# Autodesk Inventor assembly: Flywheels
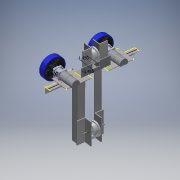
[picture p0: Inventor's stored thumbnail of the model, 180x180]
Saved by Autodesk Inventor 2017 (Build 210142000, 142)
## iProperties
Created: 2016-10-19
Part Number: Flywheels
Document SubType Name: Assembly
Designer: Aditya
Author: Aditya
## Documents named in this file (14)
- C:\Users\Aditya\Documents\GitHub\RobotuxCAD\Team Robotux 15-16 Robot Cad Assets\Flywheels.iam
- C:\Users\Aditya\Documents\GitHub\RobotuxCAD\Team Robotux 15-16 Robot Cad Assets\Flywheel w motor.iam
- C:\Users\Aditya\Documents\GitHub\RobotuxCAD\Team Robotux 15-16 Robot Cad Assets\flywheel plate.ipt
- C:\Users\Aditya\Documents\GitHub\RobotuxCAD\Team Robotux 15-16 Robot Cad Assets\Flywheel Headpiece.ipt
- C:\Users\Aditya\Documents\GitHub\RobotuxCAD\Team Robotux 15-16 Robot Cad Assets\Flywheel w motor_MIR.iam
- C:\Users\Aditya\Documents\GitHub\RobotuxCAD\Team Robotux 15-16 Robot Cad Assets\flywheel plate_MIR.ipt
- C:\Users\Aditya\Documents\GitHub\RobotuxCAD\Team Robotux 15-16 Robot Cad Assets\Long Boi.ipt
- C:\Users\Aditya\Documents\GitHub\RobotuxCAD\Team Robotux 15-16 Robot Cad Assets\Long Boi_MIR.ipt
- C:\Users\Aditya\Documents\GitHub\RobotuxCAD\Team Robotux 15-16 Robot Cad Assets\cut top wheel mout thingy.ipt
- C:\Users\Aditya\Documents\GitHub\RobotuxCAD\Team Robotux 15-16 Robot Cad Assets\Flywheel top lift wheel bracket.ipt
- C:\Users\Aditya\Documents\GitHub\RobotuxCAD\Team Robotux 15-16 Robot Cad Assets\tank tread tetrix.ipt
- C:\Users\Aditya\Documents\GitHub\RobotuxCAD\Team Robotux 15-16 Robot Cad Assets\Tetrix Parts\tetrix_739088_2013.ipt
- C:\Users\Aditya\Documents\GitHub\RobotuxCAD\Team Robotux 15-16 Robot Cad Assets\Tetrix Parts\tetrix_739091_2013.ipt
- C:\Users\Aditya\Documents\GitHub\RobotuxCAD\Team Robotux 15-16 Robot Cad Assets\Tetrix Parts\tetrix_739273_2013.ipt
## Components (22 placed, 13 different names)
1. Flywheel w motor:1 [sub-assembly] — Mate:1, Flush:1, Mate:2, Mate:46, Mate:49
2. flywheel plate:1 — Mate:1, Flush:1, Mate:2, Mate:5, Mate:7, Mate:8, Mate:11, Mate:12, Mate:16, Mate:19, Mate:45
3. Flywheel Headpiece:1 — Mate:5, Mate:6, Mate:7, Mate:8, Mate:9, Mate:10, Mate:11, Mate:12, Mate:13, Mate:14, Mate:15, Flush:3, Mate:17, Flush:4
4. Flywheel w motor_MIR:1 [sub-assembly] — Mate:3, Flush:2, Mate:4, Mate:47, Mate:48
5. flywheel plate_MIR:1 — Mate:3, Flush:2, Mate:4, Mate:6, Mate:9, Mate:10, Mate:13, Mate:14, Mate:18
6. Long Boi:1 — Mate:17, Flush:4, Mate:18, Mate:25, Flush:7, Flush:8
7. Long Boi_MIR:1 — Mate:15, Flush:3, Mate:16, Mate:26, Flush:9, Flush:10
8. cut top wheel mout thingy:1 — Mate:19, Mate:21, Flush:5, Mate:22, Mate:34, Flush:11, Mate:43, Mate:45
9. Flywheel top lift wheel bracket:1 — Mate:25, Flush:7, Flush:8, Mate:29, Mate:30
10. Flywheel top lift wheel bracket:2 — Mate:21, Flush:5, Mate:22, Mate:37, Mate:38
11. Flywheel top lift wheel bracket:3 — Mate:26, Flush:9, Flush:10, Mate:28
12. Flywheel top lift wheel bracket:4 — Mate:34, Flush:11, Mate:39, Mate:40, Mate:43
13. tank tread tetrix:1 — Mate:33
14. tank tread tetrix:2 — Mate:42
15. tetrix_739088_2013:1 — Mate:41, Mate:42
16. tetrix_739088_2013:2 — Mate:31, Mate:32, Mate:33
17. tetrix_739091_2013:1 — Mate:29, Mate:30, Mate:31
18. tetrix_739091_2013:2 — Mate:37, Mate:38, Mate:41
19. tetrix_739091_2013:3 — Mate:28, Mate:32
20. tetrix_739091_2013:4 — Mate:39, Mate:40
21. tetrix_739273_2013:1 — Mate:46, Mate:49
22. tetrix_739273_2013:2 — Mate:47, Mate:48
## Relationships (52: Mate 42, Flush 10)
- Mate:1: Flywheel w motor:1 ↔ flywheel plate:1
- Flush:1: Flywheel w motor:1 ↔ flywheel plate:1
- Mate:2: Flywheel w motor:1 ↔ flywheel plate:1
- Mate:3: Flywheel w motor_MIR:1 ↔ flywheel plate_MIR:1
- Flush:2: Flywheel w motor_MIR:1 ↔ flywheel plate_MIR:1
- Mate:4: Flywheel w motor_MIR:1 ↔ flywheel plate_MIR:1
- Mate:5: flywheel plate:1 ↔ Flywheel Headpiece:1
- Mate:6: Flywheel Headpiece:1 ↔ flywheel plate_MIR:1
- Mate:7: flywheel plate:1 ↔ Flywheel Headpiece:1
- Mate:8: flywheel plate:1 ↔ Flywheel Headpiece:1
- Mate:9: Flywheel Headpiece:1 ↔ flywheel plate_MIR:1
- Mate:10: Flywheel Headpiece:1 ↔ flywheel plate_MIR:1
- Mate:11: flywheel plate:1 ↔ Flywheel Headpiece:1
- Mate:12: flywheel plate:1 ↔ Flywheel Headpiece:1
- Mate:13: Flywheel Headpiece:1 ↔ flywheel plate_MIR:1
- Mate:14: Flywheel Headpiece:1 ↔ flywheel plate_MIR:1
- Mate:15: Flywheel Headpiece:1 ↔ Long Boi_MIR:1
- Flush:3: Flywheel Headpiece:1 ↔ Long Boi_MIR:1
- Mate:16: flywheel plate:1 ↔ Long Boi_MIR:1
- Mate:17: Flywheel Headpiece:1 ↔ Long Boi:1
- Flush:4: Flywheel Headpiece:1 ↔ Long Boi:1
- Mate:18: flywheel plate_MIR:1 ↔ Long Boi:1
- Mate:19: flywheel plate:1 ↔ cut top wheel mout thingy:1
- Mate:21: cut top wheel mout thingy:1 ↔ Flywheel top lift wheel bracket:2
- Flush:5: cut top wheel mout thingy:1 ↔ Flywheel top lift wheel bracket:2
- Mate:22: cut top wheel mout thingy:1 ↔ Flywheel top lift wheel bracket:2
- Mate:25: Long Boi:1 ↔ Flywheel top lift wheel bracket:1
- Flush:7: Long Boi:1 ↔ Flywheel top lift wheel bracket:1
- Flush:8: Long Boi:1 ↔ Flywheel top lift wheel bracket:1
- Mate:26: Long Boi_MIR:1 ↔ Flywheel top lift wheel bracket:3
- Flush:9: Long Boi_MIR:1 ↔ Flywheel top lift wheel bracket:3
- Flush:10: Long Boi_MIR:1 ↔ Flywheel top lift wheel bracket:3
- Mate:28: Flywheel top lift wheel bracket:3 ↔ tetrix_739091_2013:3
- Mate:29: Flywheel top lift wheel bracket:1 ↔ tetrix_739091_2013:1
- Mate:30: Flywheel top lift wheel bracket:1 ↔ tetrix_739091_2013:1
- Mate:31: tetrix_739088_2013:2 ↔ tetrix_739091_2013:1
- Mate:32: tetrix_739088_2013:2 ↔ tetrix_739091_2013:3
- Mate:33: tank tread tetrix:1 ↔ tetrix_739088_2013:2
- Mate:34: cut top wheel mout thingy:1 ↔ Flywheel top lift wheel bracket:4
- Flush:11: cut top wheel mout thingy:1 ↔ Flywheel top lift wheel bracket:4
- Mate:37: Flywheel top lift wheel bracket:2 ↔ tetrix_739091_2013:2
- Mate:38: Flywheel top lift wheel bracket:2 ↔ tetrix_739091_2013:2
- Mate:39: Flywheel top lift wheel bracket:4 ↔ tetrix_739091_2013:4
- Mate:40: Flywheel top lift wheel bracket:4 ↔ tetrix_739091_2013:4
- Mate:41: tetrix_739088_2013:1 ↔ tetrix_739091_2013:2
- Mate:42: tank tread tetrix:2 ↔ tetrix_739088_2013:1
- Mate:43: cut top wheel mout thingy:1 ↔ Flywheel top lift wheel bracket:4
- Mate:45: flywheel plate:1 ↔ cut top wheel mout thingy:1
- Mate:46: Flywheel w motor:1 ↔ tetrix_739273_2013:1
- Mate:47: Flywheel w motor_MIR:1 ↔ tetrix_739273_2013:2
- Mate:48: Flywheel w motor_MIR:1 ↔ tetrix_739273_2013:2
- Mate:49: Flywheel w motor:1 ↔ tetrix_739273_2013:1
